# Autodesk Inventor assembly: Shoulder
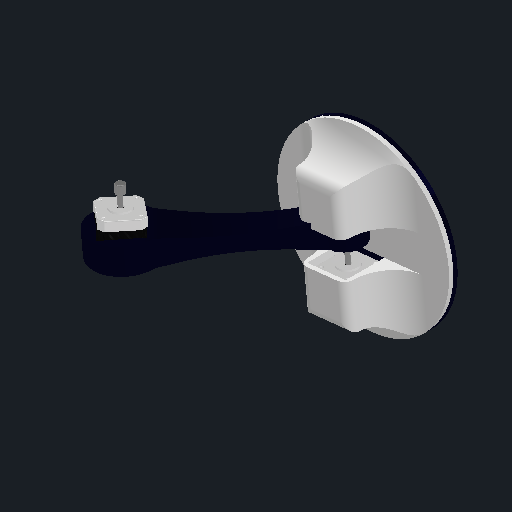
[picture p0: Inventor's stored thumbnail of the model, 512x512]
Saved by Autodesk Inventor 2023 (Build 270158000, 158)
## iProperties
Created: 2023-04-07
Part Number: Shoulder
Document SubType Name: Assembly
Designer: vatdu
Author: vatdu
## Documents named in this file (5)
- C:\Users\vatdu\Desktop\CRYSTAL MARK II\Shoulder\Shoulder.iam
- C:\Users\vatdu\Desktop\CRYSTAL MARK II\Shoulder\Rotating Plate.ipt
- C:\Users\vatdu\Desktop\CRYSTAL MARK II\Components\Stepper Motor.ipt
- C:\Users\vatdu\Desktop\CRYSTAL MARK II\Shoulder\Arm Extention.ipt
- C:\Users\vatdu\Desktop\CRYSTAL MARK II\Shoulder\Motor Cover V2.ipt
## Components (6 placed, 4 different names)
1. Rotating Plate:1 — Rotational:2
2. Arm Extention:1 — Rigid:1, Rotational:1, Rigid:4
3. Stepper Motor:2 — Rigid:1, Rigid:4
4. Motor Cover V2:1 — Rigid:2, Rigid:3, Rotational:2
5. Stepper Motor:3 — Rigid:3, Rotational:1
6. Stepper Motor:4 — Rigid:2
## Relationships (6: WeldJoint 4, RevoluteJoint 2)
- Rigid:1 [WeldJoint]: Arm Extention:1 ↔ Stepper Motor:2
- Rigid:2 [WeldJoint]: Motor Cover V2:1 ↔ Stepper Motor:4
- Rigid:3 [WeldJoint]: Motor Cover V2:1 ↔ Stepper Motor:3
- Rotational:1 [RevoluteJoint]: Arm Extention:1 ↔ Stepper Motor:3
- Rotational:2 [RevoluteJoint]: Rotating Plate:1 ↔ Motor Cover V2:1
- Rigid:4 [WeldJoint]: Arm Extention:1 ↔ Stepper Motor:2
